# Autodesk Inventor assembly: Pancake Pneumatic
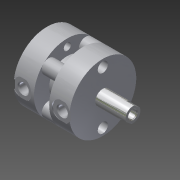
[picture p0: Inventor's stored thumbnail of the model, 180x180]
Saved by Autodesk Inventor 2014 SP1 (Build 180222100, 222)
## iProperties
Created: 2013-06-28
Part Number: Pancake Pneumatic
Document SubType Name: Assembly
Designer: mvarma
Mass: 29.5482 g
Surface Area: 81.5149 cm^2
Volume: 11.068 cm^3
Density: 2.6697 g/cm^3
Author: mvarma
## Documents named in this file (7)
- C:\Users\Rauhul Varma\Desktop\GRT 2013-2014 Designs\Build Gearbox Mark 1\Pneumatic\Pancake Pneumatic.iam
- C:\Users\Rauhul Varma\Desktop\GRT 2013-2014 Designs\Build Gearbox Mark 1\Pneumatic\Pneumatic Parts\Axle.ipt
- C:\Users\Rauhul Varma\Desktop\GRT 2013-2014 Designs\Build Gearbox Mark 1\Pneumatic\Pneumatic Parts\Bore.ipt
- C:\Users\Rauhul Varma\Desktop\GRT 2013-2014 Designs\Build Gearbox Mark 1\Pneumatic\Pneumatic Parts\Cylinder.ipt
- C:\Users\Rauhul Varma\Desktop\GRT 2013-2014 Designs\Build Gearbox Mark 1\Pneumatic\Pneumatic Parts\Front Mount.ipt
- C:\Users\Rauhul Varma\Desktop\GRT 2013-2014 Designs\Build Gearbox Mark 1\Pneumatic\Pneumatic Parts\Rear Mount.ipt
- C:\Users\Rauhul Varma\Desktop\GRT 2013-2014 Designs\Build Gearbox Mark 1\Pneumatic\Pneumatic Parts\Spacer.ipt
## Components (9 placed, 6 different names)
1. Axle:1 — Mate:11, Flush:1
2. Bore:1 — Mate:11, Flush:1, Mate:12, Mate:13
3. Cylinder:1 — Mate:9, Mate:10, Mate:12
4. Front Mount:1 — Mate:14, Mate:15, Mate:16
5. Rear Mount:1 — Mate:1, Mate:2, Mate:3, Mate:4, Mate:5, Mate:6, Mate:7, Mate:8, Mate:9, Mate:10, Mate:13, Mate:14
6. Spacer:1 — Mate:2, Mate:7
7. Spacer:2 — Mate:4, Mate:8
8. Spacer:3 — Mate:3, Mate:6, Mate:15, Mate:16
9. Spacer:4 — Mate:1, Mate:5
## Relationships (17: Mate 16, Flush 1)
- Mate:1: Rear Mount:1 ↔ Spacer:4
- Mate:2: Rear Mount:1 ↔ Spacer:1
- Mate:3: Rear Mount:1 ↔ Spacer:3
- Mate:4: Rear Mount:1 ↔ Spacer:2
- Mate:5: Rear Mount:1 ↔ Spacer:4
- Mate:6: Rear Mount:1 ↔ Spacer:3
- Mate:7: Rear Mount:1 ↔ Spacer:1
- Mate:8: Rear Mount:1 ↔ Spacer:2
- Mate:9: Cylinder:1 ↔ Rear Mount:1
- Mate:10: Cylinder:1 ↔ Rear Mount:1
- Mate:11: Axle:1 ↔ Bore:1
- Flush:1: Axle:1 ↔ Bore:1
- Mate:12: Bore:1 ↔ Cylinder:1
- Mate:13: Bore:1 ↔ Rear Mount:1
- Mate:14: Front Mount:1 ↔ Rear Mount:1
- Mate:15: Front Mount:1 ↔ Spacer:3
- Mate:16: Front Mount:1 ↔ Spacer:3
